# Autodesk Inventor assembly: Chair-Side-Mir
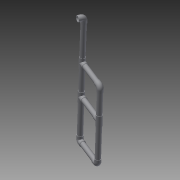
[picture p0: Inventor's stored thumbnail of the model, 180x180]
Saved by Autodesk Inventor 2015 (Build 190159000, 159)
## iProperties
Created: 2015-05-01
Part Number: Chair-Side-Mir
Document SubType Name: Assembly
Designer: 1750019
Author: 1750019
## Documents named in this file (5)
- R:\VD Proj\Chair-Side-Mir.iam
- R:\VD Proj\MCMasterCarr\Imported Components\90 ELBOW - 4880K260\90 ELBOW - 4880K260.ipt
- R:\VD Proj\Generic 1ft Segment.ipt
- R:\VD Proj\18 in Seg.ipt
- R:\VD Proj\MCMasterCarr\Imported Components\TEE - 4880K460\TEE - 4880K460.ipt
## Components (15 placed, 4 different names)
1. 90 ELBOW - 4880K260:1 — Rigid:2, Rigid:3
2. Generic 1ft Segment:1 — Rigid:1, Rigid:3
3. 90 ELBOW - 4880K260:2 — Rigid:1, Rigid:8
4. 18 in Seg:1 — Rigid:2, Rigid:5
5. 18 in Seg:2 — Rigid:6, Rigid:8
6. TEE - 4880K460:1 — Rigid:5, Rigid:9, Rigid:11
7. TEE - 4880K460:2 — Rigid:6, Rigid:10
8. Generic 1ft Segment:2 — Rigid:9
9. Generic 1ft Segment:3 — Rigid:11, Rigid:12
10. Generic 1ft Segment:4 — Rigid:10, Rigid:14
11. 90 ELBOW - 4880K260:3 — Rigid:12, Rigid:13
12. Generic 1ft Segment:5 — Rigid:13, Angle:1
13. 18 in Seg:3 — Rigid:15, Insert:1
14. TEE - 4880K460:3 — Rigid:14, Rigid:15
15. 90 ELBOW - 4880K260:4 — Insert:1, Angle:1
## Relationships (15: WeldJoint 13, Insert 1, Angle 1)
- Rigid:1 [WeldJoint]: Generic 1ft Segment:1 ↔ 90 ELBOW - 4880K260:2
- Rigid:2 [WeldJoint]: 90 ELBOW - 4880K260:1 ↔ 18 in Seg:1
- Rigid:3 [WeldJoint]: 90 ELBOW - 4880K260:1 ↔ Generic 1ft Segment:1
- Rigid:5 [WeldJoint]: 18 in Seg:1 ↔ TEE - 4880K460:1
- Rigid:6 [WeldJoint]: 18 in Seg:2 ↔ TEE - 4880K460:2
- Rigid:8 [WeldJoint]: 90 ELBOW - 4880K260:2 ↔ 18 in Seg:2
- Rigid:9 [WeldJoint]: TEE - 4880K460:1 ↔ Generic 1ft Segment:2
- Rigid:10 [WeldJoint]: TEE - 4880K460:2 ↔ Generic 1ft Segment:4
- Rigid:11 [WeldJoint]: TEE - 4880K460:1 ↔ Generic 1ft Segment:3
- Rigid:12 [WeldJoint]: Generic 1ft Segment:3 ↔ 90 ELBOW - 4880K260:3
- Rigid:13 [WeldJoint]: 90 ELBOW - 4880K260:3 ↔ Generic 1ft Segment:5
- Rigid:14 [WeldJoint]: Generic 1ft Segment:4 ↔ TEE - 4880K460:3
- Rigid:15 [WeldJoint]: 18 in Seg:3 ↔ TEE - 4880K460:3
- Insert:1: 18 in Seg:3 ↔ 90 ELBOW - 4880K260:4
- Angle:1 (-90 deg): Generic 1ft Segment:5 ↔ 90 ELBOW - 4880K260:4
